# Autodesk Inventor assembly: primer pieza
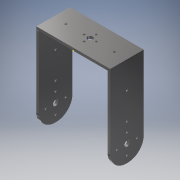
[picture p0: Inventor's stored thumbnail of the model, 180x180]
Saved by Autodesk Inventor 2018 (Build 220112000, 112)
## iProperties
Created: 2019-04-02
Part Number: primer pieza
Material: Genérico
Document SubType Name: Assembly
Designer: Victor Hernandez
Author: Victor Hernandez
## Documents named in this file (3)
- C:\Users\Victor Hernandez\Desktop\Quinto Cuatrimestre\Garabito\robot\primer pieza.iam
- C:\Users\Victor Hernandez\Desktop\Quinto Cuatrimestre\Garabito\robot\frontal.ipt
- C:\Users\Victor Hernandez\Desktop\Quinto Cuatrimestre\Garabito\robot\laterales.ipt
## Components (3 placed, 2 different names)
1. frontal:1 — Coincidencia:1, Coincidencia:2, Coincidencia:3
2. laterales:1 — Coincidencia:1, Coincidencia:3
3. laterales:2 — Coincidencia:2
## Relationships (3: Mate 3)
- Coincidencia:1 [Mate]: frontal:1 ↔ laterales:1
- Coincidencia:2 [Mate]: frontal:1 ↔ laterales:2
- Coincidencia:3 [Mate]: frontal:1 ↔ laterales:1
